# Autodesk Inventor assembly: top-idler
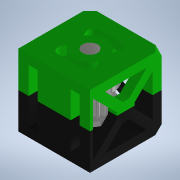
[picture p0: Inventor's stored thumbnail of the model, 180x180]
Saved by Autodesk Inventor 2020.4 (Build 244396000, 396)
## iProperties
Created: 2021-04-07
Part Number: top-idler
Document SubType Name: Assembly
Designer: AOB
Mass: 12.0264 g
Surface Area: 79.1486 cm^2
Volume: 6.84072 cm^3
Density: 1.75805 g/cm^3
Author: AOB
## Documents named in this file (4)
- C:\Users\marti\Documents\Inventor\ProjectBoron\Boron Ultima\top-idler.iam
- C:\Users\marti\Documents\Inventor\ProjectBoron\Boron Ultima\top-idler V2.ipt
- C:\Users\marti\Documents\Inventor\ProjectBoron\Boron Ultima\5mm short(24mm) shaft.ipt
- C:\Users\marti\Documents\Inventor\ProjectBoron\Boron Ultima\GT2 20T Idler Gates.ipt
## Components (4 placed, 3 different names)
1. top-idler V2:1 — Flush:1, Flush:2, Rigid:1
2. top-idler V2:2 — Flush:1, Flush:2, Rigid:1, Mate:1, Flush:3, Mate:3
3. 5mm short(24mm) shaft:1 — Mate:1, Flush:3, Mate:2
4. GT2 20T Idler Gates:1 — Mate:2, Mate:3
## Relationships (7: Flush 3, Mate 3, WeldJoint 1)
- Flush:1: top-idler V2:1 ↔ top-idler V2:2
- Flush:2: top-idler V2:1 ↔ top-idler V2:2
- Rigid:1 [WeldJoint]: top-idler V2:1 ↔ top-idler V2:2
- Mate:1: top-idler V2:2 ↔ 5mm short(24mm) shaft:1
- Flush:3: top-idler V2:2 ↔ 5mm short(24mm) shaft:1
- Mate:2: 5mm short(24mm) shaft:1 ↔ GT2 20T Idler Gates:1
- Mate:3 (3.5 mm): top-idler V2:2 ↔ GT2 20T Idler Gates:1
